# Autodesk Inventor assembly: frame
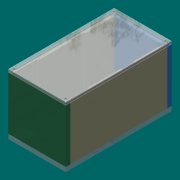
[picture p0: Inventor's stored thumbnail of the model, 180x180]
Saved by Autodesk Inventor 2016 (Build 200138000, 138)
## iProperties
Created: 2015-10-13
Part Number: frame
Document SubType Name: Assembly
Designer: Sawaiz
Author: Sawaiz
## Documents named in this file (10)
- C:\Users\Sawaiz\OneDrive\projects\modularRICH\frame\frame.iam
- C:\Users\Sawaiz\OneDrive\projects\modularRICH\frame\leftSide.ipt
- C:\Users\Sawaiz\OneDrive\projects\modularRICH\frame\rightSide.ipt
- C:\Users\Sawaiz\OneDrive\projects\modularRICH\frame\back.ipt
- C:\Users\Sawaiz\OneDrive\projects\modularRICH\frame\bottom.ipt
- C:\Users\Sawaiz\OneDrive\projects\modularRICH\frame\front.ipt
- C:\Users\Sawaiz\OneDrive\projects\modularRICH\frame\top.ipt
- C:\Users\Sawaiz\OneDrive\projects\modularRICH\frame\4-40x0.5in.ipt
- C:\Users\Sawaiz\OneDrive\projects\modularRICH\frame\topORing.ipt
- C:\Users\Sawaiz\OneDrive\projects\modularRICH\modularRICH.xlsx
## Components (11 placed, 8 different names)
1. leftSide:1 — Flush:1, Flush:2, Flush:9, Flush:10
2. rightSide:1 — Flush:1, Flush:2, Flush:3, Flush:4, Flush:5, Mate:2, Flush:8, Mate:3
3. back:1 — Flush:4, Flush:8, Mate:3, Flush:11
4. bottom:1 — Flush:6, Mate:1, Flush:7
5. front:1 — Flush:3, Flush:5, Flush:6, Mate:1, Flush:7, Mate:2, Flush:9, Mate:11
6. top:1 — Flush:10, Flush:11, Mate:4, Mate:5, Mate:6, Mate:7, Flush:12, Flush:13, Flush:14, Flush:15, Mate:8, Mate:9, Mate:10, Mate:11
7. 4-40x0.5in:1 — Mate:4, Flush:15
8. 4-40x0.5in:2 — Mate:7, Flush:12
9. 4-40x0.5in:3 — Mate:6, Flush:13
10. 4-40x0.5in:4 — Mate:5, Flush:14
11. topORing:1 — Mate:8, Mate:9, Mate:10
## Relationships (26: Flush 15, Mate 11)
- Flush:1: leftSide:1 ↔ rightSide:1
- Flush:2: leftSide:1 ↔ rightSide:1
- Flush:3: rightSide:1 ↔ front:1
- Flush:4: rightSide:1 ↔ back:1
- Flush:5: rightSide:1 ↔ front:1
- Flush:6: bottom:1 ↔ front:1
- Mate:1: bottom:1 ↔ front:1
- Flush:7: bottom:1 ↔ front:1
- Mate:2: rightSide:1 ↔ front:1
- Flush:8: rightSide:1 ↔ back:1
- Mate:3: rightSide:1 ↔ back:1
- Flush:9: leftSide:1 ↔ front:1
- Flush:10: leftSide:1 ↔ top:1
- Flush:11: back:1 ↔ top:1
- Mate:4: top:1 ↔ 4-40x0.5in:1
- Mate:5: top:1 ↔ 4-40x0.5in:4
- Mate:6: top:1 ↔ 4-40x0.5in:3
- Mate:7: top:1 ↔ 4-40x0.5in:2
- Flush:12: top:1 ↔ 4-40x0.5in:2
- Flush:13: top:1 ↔ 4-40x0.5in:3
- Flush:14: top:1 ↔ 4-40x0.5in:4
- Flush:15: top:1 ↔ 4-40x0.5in:1
- Mate:8: top:1 ↔ topORing:1
- Mate:9: top:1 ↔ topORing:1
- Mate:10: top:1 ↔ topORing:1
- Mate:11: front:1 ↔ top:1
## Named parameters: acrylicThickness = 6.35 mm, aerogelThickness = 30 mm, height = 101.6 mm, width = 101.6 mm, depth = 203.2 mm, mirrorAngle = 5 deg, detectorWidth = 52 mm, detectorHeight = 52 mm, mirrorThickness = 3.175 mm, fresnelThickness = 0.1 mm, grooveDensity = 100, focalLength = 76.2 mm, ior = 1.49, centerThickness = 1.524 mm, fresnelAngle = 90 deg, fresnelEffectiveDiameter = 76.2 mm, mirrorSuppourtWidth = 38.1 mm, backGrooveBit = 4.8006 mm, sensorHolderWidth = 88.9 mm, sensorHolderSensorWidth = 53.975 mm, sensorHolderSesnorHeight = 53.975 mm, sensorHolderHeight = 88.9 mm, sensorHolderSensorHeight = 53.975 mm, sensorHolderORingGroove = 3.175 mm, sensorHolderORing = 3.175 mm, sensorHolderFlushORingID = 304.8 mm, sensorHolderFlushORing = 3.175 mm, frontBackORingID = 419.1 mm, oRingWidth = 1.5875 mm, sensorHolderORingID = 203.2 mm, topBottomHorizontalMirrorGroove = 12.7 mm, backMirrorGroove = 6.35 mm, mirrorGroove = 19.05 mm, compressionPercent = 40, fresnelChamfer = 6.35 mm, mirrorGrooveFillet = 6.35 mm, mirrorGrooveDrill = 6.35 mm, mirrorGrooveMill = 3.175 mm, fresnelMirrorChamfer = 6.35 mm, detectorOpeningHeight = 76.2 mm, detectorOpeningWidth = 76.2 mm, sensorHolderDepth = 19.05 mm, frameAcrylicThickness = 9.525 mm, internalAcrylicThicnkess = 6.35 mm, aerogelWidth = 101.6 mm, aerogelHeight = 101.6 mm, internalAcrylicThickness = 6.35 mm
